# Autodesk Inventor assembly: Finger_clean
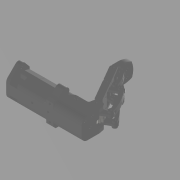
[picture p0: Inventor's stored thumbnail of the model, 180x180]
Saved by Autodesk Inventor 2016 (Build 200138000, 138)
## iProperties
Created: 2015-01-03
Part Number: Finger_clean
Document SubType Name: Assembly
Designer: 4ndreas
Mass: 93.4744 g
Surface Area: 487.806 cm^2
Volume: 80.2696 cm^3
Density: 1.16451 g/cm^3
Author: 4ndreas
## Documents named in this file (15)
- C:\Users\4ndreas\Documents\Inventor\RobotARM v2\Gripper V1\Finger_clean.iam
- C:\Users\4ndreas\Documents\Inventor\RobotARM v2\Gripper V1\schnecke.ipt
- C:\Users\4ndreas\Documents\Inventor\RobotARM v2\Gripper V1\DC-Motor_12V_60U-min.ipt
- C:\Users\4ndreas\Documents\Inventor\RobotARM v2\Gripper V1\FingerPartA.ipt
- C:\Users\4ndreas\Documents\Inventor\RobotARM v2\Gripper V1\FingerPartB.ipt
- C:\Users\4ndreas\Documents\Inventor\RobotARM v2\Gripper V1\Hebel_Basis.ipt
- C:\Users\4ndreas\Documents\Inventor\RobotARM v2\Gripper V1\Hebel_Basis 2.ipt
- C:\Users\4ndreas\Documents\Inventor\RobotARM v2\Gripper V1\FingerMount_Mitte.ipt
- C:\Users\4ndreas\Documents\Inventor\RobotARM v2\Gripper V1\FingerTipp_middle.ipt
- C:\Users\4ndreas\Documents\Inventor\RobotARM v2\Gripper V1\deckel_mitte copy.ipt
- C:\Users\4ndreas\Documents\Inventor\RobotARM v2\Gripper V1\FingerTip_joint _v2.ipt
- C:\Users\4ndreas\Documents\Inventor\RobotARM v2\Gripper V1\3_hebenMount_2_dual.ipt
- C:\Users\4ndreas\Documents\Inventor\RobotARM v2\Gripper V1\FingerTip_Mount dual.ipt
- C:\Users\4ndreas\Documents\Inventor\RobotARM v2\Gripper V1\Hebel_B dual.ipt
- C:\Users\4ndreas\Documents\Inventor\RobotARM v2\Gripper V1\Hebel_dual.ipt
## Components (16 placed, 14 different names)
1. FingerMount_Mitte:1 — Passend:2, Passend:3, Passend:6, Passend:12, Passend:13, Passend:17, Winkel:1, Winkel:2, Winkel:3, Passend:19, Passend:20, Passend:21
2. deckel_mitte copy:1 — Passend:19, Passend:20, Passend:21
3. schnecke:1 — Passend:4
4. DC-Motor_12V_60U-min:1 — Passend:1, Passend:3, Winkel:2
5. FingerPartA:1 — Passend:6, Passend:8, Passend:9, Passend:12, Passend:14, Fluchtend:1, Passend:15
6. FingerPartB:1 — Passend:8, Passend:9, Passend:10, Passend:11, Fluchtend:1, Passend:22, Passend:24, Passend:26, Passend:27, Passend:28
7. FingerTipp_middle:1 — Passend:10, Passend:11, Fluchtend:3, Passend:23, Passend:29, Passend:31
8. Hebel_Basis:1 — Passend:13, Passend:14, Passend:16, Passend:18, Passend:41, Passend:42
9. Hebel_Basis 2:1 — Passend:15, Passend:16, Passend:38, Passend:39
10. FingerTip_joint _v2:1 — Passend:22, Passend:23, Passend:34
11. 3_hebenMount_2_dual:1 — Passend:26, Passend:28, Passend:33, Passend:36, Passend:37
12. FingerTip_Mount dual:1 — Passend:24, Passend:27, Passend:32, Passend:40
13. Hebel_B dual:1 — Passend:29, Passend:31, Passend:32
14. Hebel_B dual:2 — Passend:33, Passend:34, Passend:36
15. Hebel_dual:1 — Passend:37, Passend:38, Passend:39
16. Hebel_dual:2 — Passend:40, Passend:41, Passend:42
## Relationships (43: Mate 37, Flush 3, Angle 3)
- Passend:1 [Mate]: DC-Motor_12V_60U-min:1
- Passend:2 [Mate]: FingerMount_Mitte:1
- Passend:3 [Mate]: FingerMount_Mitte:1 ↔ DC-Motor_12V_60U-min:1
- Passend:4 [Mate]: schnecke:1
- Passend:6 [Mate]: FingerMount_Mitte:1 ↔ FingerPartA:1
- Passend:8 [Mate]: FingerPartA:1 ↔ FingerPartB:1
- Passend:9 [Mate]: FingerPartA:1 ↔ FingerPartB:1
- Passend:10 [Mate]: FingerPartB:1 ↔ FingerTipp_middle:1
- Passend:11 [Mate]: FingerPartB:1 ↔ FingerTipp_middle:1
- Passend:12 [Mate]: FingerMount_Mitte:1 ↔ FingerPartA:1
- Passend:13 [Mate]: FingerMount_Mitte:1 ↔ Hebel_Basis:1
- Passend:14 [Mate]: FingerPartA:1 ↔ Hebel_Basis:1
- Fluchtend:1 [Flush]: FingerPartA:1 ↔ FingerPartB:1
- Passend:15 [Mate]: FingerPartA:1 ↔ Hebel_Basis 2:1
- Passend:16 [Mate]: Hebel_Basis:1 ↔ Hebel_Basis 2:1
- Passend:17 [Mate]: FingerMount_Mitte:1
- Winkel:1 [Angle] (0 deg): FingerMount_Mitte:1
- Winkel:2 [Angle] (0 deg): FingerMount_Mitte:1 ↔ DC-Motor_12V_60U-min:1
- Passend:18 [Mate]: Hebel_Basis:1
- Winkel:3 [Angle] (90 deg): FingerMount_Mitte:1
- Fluchtend:2 [Flush] (36.5 mm)
- Fluchtend:3 [Flush]: FingerTipp_middle:1
- Passend:19 [Mate]: FingerMount_Mitte:1 ↔ deckel_mitte copy:1
- Passend:20 [Mate]: FingerMount_Mitte:1 ↔ deckel_mitte copy:1
- Passend:21 [Mate]: FingerMount_Mitte:1 ↔ deckel_mitte copy:1
- Passend:22 [Mate]: FingerPartB:1 ↔ FingerTip_joint _v2:1
- Passend:23 [Mate]: FingerTipp_middle:1 ↔ FingerTip_joint _v2:1
- Passend:24 [Mate]: FingerPartB:1 ↔ FingerTip_Mount dual:1
- Passend:26 [Mate]: FingerPartB:1 ↔ 3_hebenMount_2_dual:1
- Passend:27 [Mate]: FingerPartB:1 ↔ FingerTip_Mount dual:1
- Passend:28 [Mate]: FingerPartB:1 ↔ 3_hebenMount_2_dual:1
- Passend:29 [Mate]: FingerTipp_middle:1 ↔ Hebel_B dual:1
- Passend:31 [Mate]: FingerTipp_middle:1 ↔ Hebel_B dual:1
- Passend:32 [Mate]: FingerTip_Mount dual:1 ↔ Hebel_B dual:1
- Passend:33 [Mate]: 3_hebenMount_2_dual:1 ↔ Hebel_B dual:2
- Passend:34 [Mate]: FingerTip_joint _v2:1 ↔ Hebel_B dual:2
- Passend:36 [Mate]: 3_hebenMount_2_dual:1 ↔ Hebel_B dual:2
- Passend:37 [Mate]: 3_hebenMount_2_dual:1 ↔ Hebel_dual:1
- Passend:38 [Mate]: Hebel_Basis 2:1 ↔ Hebel_dual:1
- Passend:39 [Mate]: Hebel_Basis 2:1 ↔ Hebel_dual:1
- Passend:40 [Mate]: FingerTip_Mount dual:1 ↔ Hebel_dual:2
- Passend:41 [Mate]: Hebel_Basis:1 ↔ Hebel_dual:2
- Passend:42 [Mate]: Hebel_Basis:1 ↔ Hebel_dual:2
